# Autodesk Inventor assembly: leg_right
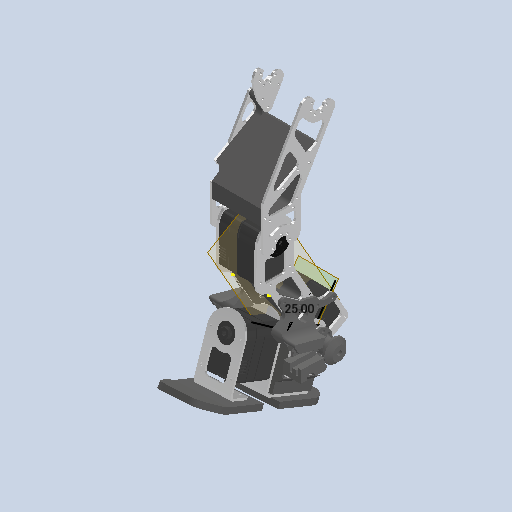
[picture p0: Inventor's stored thumbnail of the model, 512x512]
Saved by Autodesk Inventor 2026.1 (Build 301233020, 233B)
## iProperties
Created: 2024-10-11
Part Number: leg_right
Document SubType Name: Assembly
Designer: hibik
Author: hibik
## Documents named in this file (9)
- C:\Users\hibik\Documents\Robomech\HR\Eglantyne_mark2\hard\leg\leg_right.iam
- C:\Users\hibik\Documents\Robomech\HR\Eglantyne_mark2\hard\leg\leg_upper_right.iam
- C:\Users\hibik\Documents\Robomech\HR\Eglantyne_mark2\hard\leg\leg_under.iam
- C:\Users\hibik\Documents\Robomech\HR\Eglantyne_mark2\hard\leg\toe.iam
- C:\Users\hibik\Documents\Robomech\HR\Eglantyne_mark2\hard\leg\spring_setter\axis.ipt
- C:\Users\hibik\Documents\Robomech\HR\Eglantyne_mark2\hard\leg\spring_setter\setter_upper.ipt
- C:\Users\hibik\Documents\Robomech\HR\Eglantyne_mark2\hard\leg\spring_setter\axis_MIR.ipt
- C:\Users\hibik\Documents\Robomech\HR\Eglantyne_mark2\hard\leg\spring_setter\setter_upper_MIR.ipt
- C:\Users\hibik\Documents\Robomech\HR\Eglantyne_mark2\hard\leg\spring_setter\cover.ipt
## Components (9 placed, 8 different names)
1. leg_upper_right:1 [sub-assembly] — 挿入:1
2. leg_under:1 [sub-assembly] — 挿入:1, 挿入:2, 挿入:5, 角度:1
3. toe:1 [sub-assembly] — 挿入:2, 挿入:3, 挿入:4
4. axis:1 — 挿入:3, 挿入:4, メイト:1, 挿入:6
5. setter_upper:1 — 挿入:5, メイト:1, 角度:1
6. axis_MIR:1 — メイト:2, 挿入:7
7. setter_upper_MIR:1 — メイト:2
8. cover:1 — 挿入:6
9. cover:2 — 挿入:7
## Relationships (10: Insert 7, Mate 2, Angle 1)
- 挿入:1 [Insert]: leg_upper_right:1 ↔ leg_under:1
- 挿入:2 [Insert]: leg_under:1 ↔ toe:1
- 挿入:3 [Insert]: toe:1 ↔ axis:1
- 挿入:4 [Insert]: toe:1 ↔ axis:1
- 挿入:5 [Insert]: leg_under:1 ↔ setter_upper:1
- メイト:1 [Mate]: axis:1 ↔ setter_upper:1
- メイト:2 [Mate]: axis_MIR:1 ↔ setter_upper_MIR:1
- 挿入:6 [Insert]: axis:1 ↔ cover:1
- 挿入:7 [Insert]: axis_MIR:1 ↔ cover:2
- 角度:1 [Angle] (0 deg): leg_under:1 ↔ setter_upper:1
